# Autodesk Inventor assembly: Ensamble con TuboBP
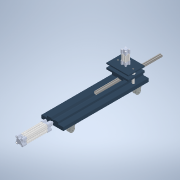
[picture p0: Inventor's stored thumbnail of the model, 180x180]
Saved by Autodesk Inventor 2021 (Build 250183000, 183)
## iProperties
Created: 2020-01-15
Part Number: Ensamble con TuboBP
Document SubType Name: Assembly
Designer: Nelson
Sending System: SolidWorks 2020
Last Author: Micro
Last Saved: 2020-01-16
Author: Nelson
## Documents named in this file (8)
- D:\Nelson\Documentos\Inventor\PrensaHidraulica_Automatizada\Ensamble con TuboBP.iam
- Prensa_Hidraulica.iam
- D:\Nelson\Documentos\Inventor\PrensaHidraulica_Automatizada\Ensamble Mecanismo cilindro.iam
- D:\Nelson\Documentos\Inventor\PrensaHidraulica_Automatizada\Barra_5-8_950.ipt
- D:\Nelson\Documentos\Inventor\PrensaHidraulica_Automatizada\Barra_5-8_400.ipt
- D:\Nelson\Documentos\Inventor\PrensaHidraulica_Automatizada\04893142.iam
- D:\Nelson\Documentos\Inventor\PrensaHidraulica_Automatizada\04303733.ipt
- D:\Nelson\Documentos\Inventor\PrensaHidraulica_Automatizada\Barra_1_1-8_600_BP.ipt
## Components (10 placed, 6 different names)
1. Ensamble mecanismo cilindro:1 [sub-assembly] — Tangent:10, Tangent:11, Tangent:14, Tangent:15, Flush:17, Mate:104, Mate:105, Flush:22, Mate:144, Flush:23, Flush:24, Flush:25, Mate:145, Flush:26, Flush:27, Mate:146, Tangent:16, Tangent:17, Mate:147
2. Barra_5-8_950:1 — Tangent:10, Tangent:11
3. Barra_5-8_400:1 — Tangent:14, Tangent:15, Flush:17
4. 04893142:2 [sub-assembly] — Mate:104, Mate:105, Flush:18, Flush:19, Mate:142, Flush:20, Mate:143, Flush:21
5. 04303733:1 — Flush:18, Flush:19, Mate:142
6. 04303733:2 — Flush:20, Mate:143, Flush:21
7. 04303733:5 — Flush:22, Mate:144, Flush:23
8. 04303733:6 — Flush:24, Flush:25, Mate:145
9. 04303733:7 — Flush:26, Flush:27, Mate:146
10. Barra_1_1-8_600_BP:1 — Tangent:16, Tangent:17, Mate:147
## Relationships (25: Flush 11, Mate 8, Tangent 6)
- Tangent:10: Ensamble mecanismo cilindro:1 ↔ Barra_5-8_950:1
- Tangent:11: Ensamble mecanismo cilindro:1 ↔ Barra_5-8_950:1
- Tangent:14: Ensamble mecanismo cilindro:1 ↔ Barra_5-8_400:1
- Tangent:15: Ensamble mecanismo cilindro:1 ↔ Barra_5-8_400:1
- Flush:17 (-214.3 mm): Ensamble mecanismo cilindro:1 ↔ Barra_5-8_400:1
- Mate:104: Ensamble mecanismo cilindro:1 ↔ 04893142:2
- Mate:105: Ensamble mecanismo cilindro:1 ↔ 04893142:2
- Flush:18 (11 mm): 04893142:2 ↔ 04303733:1
- Flush:19: 04893142:2 ↔ 04303733:1
- Mate:142 (0.35 mm): 04893142:2 ↔ 04303733:1
- Flush:20: 04893142:2 ↔ 04303733:2
- Mate:143 (0.35 mm): 04893142:2 ↔ 04303733:2
- Flush:21 (11 mm): 04893142:2 ↔ 04303733:2
- Flush:22: Ensamble mecanismo cilindro:1 ↔ 04303733:5
- Mate:144 (0.35 mm): Ensamble mecanismo cilindro:1 ↔ 04303733:5
- Flush:23 (10.5 mm): Ensamble mecanismo cilindro:1 ↔ 04303733:5
- Flush:24: Ensamble mecanismo cilindro:1 ↔ 04303733:6
- Flush:25 (24.1 mm): Ensamble mecanismo cilindro:1 ↔ 04303733:6
- Mate:145 (0.35 mm): Ensamble mecanismo cilindro:1 ↔ 04303733:6
- Flush:26: Ensamble mecanismo cilindro:1 ↔ 04303733:7
- Flush:27 (10.5 mm): Ensamble mecanismo cilindro:1 ↔ 04303733:7
- Mate:146 (0.35 mm): Ensamble mecanismo cilindro:1 ↔ 04303733:7
- Tangent:16: Ensamble mecanismo cilindro:1 ↔ Barra_1_1-8_600_BP:1
- Tangent:17: Ensamble mecanismo cilindro:1 ↔ Barra_1_1-8_600_BP:1
- Mate:147 (-385.7 mm): Ensamble mecanismo cilindro:1 ↔ Barra_1_1-8_600_BP:1
